# Autodesk Inventor assembly: Assembly1
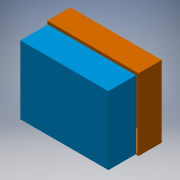
[picture p0: Inventor's stored thumbnail of the model, 180x180]
Saved by Autodesk Inventor 2016 (Build 200138000, 138)
## iProperties
Created: 2016-02-20
Part Number: Assembly1
Document SubType Name: Assembly
Designer: Róbert
Author: Róbert
## Documents named in this file (5)
- C:\Users\Róbert\Desktop\Mechatronics-2016.git\trunk\Inventor\Assembly1.iam
- C:\Users\Róbert\Desktop\Mechatronics-2016.git\trunk\Inventor\veggur_lok.ipt
- C:\Users\Róbert\Desktop\Mechatronics-2016.git\trunk\Inventor\toppur.ipt
- C:\Users\Róbert\Desktop\Mechatronics-2016.git\trunk\Inventor\botn.ipt
- C:\Users\Róbert\Desktop\Mechatronics-2016.git\trunk\Inventor\veggur.ipt
## Components (4 placed, 4 different names)
1. veggur_lok:1 — Mate:1, Flush:1, Flush:2, Mate:3
2. toppur:1 — Mate:1, Flush:1, Flush:2
3. botn:1 — Mate:2, Flush:3, Flush:4
4. veggur:1 — Mate:2, Flush:3, Flush:4, Mate:3
## Relationships (7: Flush 4, Mate 3)
- Mate:1: veggur_lok:1 ↔ toppur:1
- Flush:1: veggur_lok:1 ↔ toppur:1
- Flush:2: veggur_lok:1 ↔ toppur:1
- Mate:2: botn:1 ↔ veggur:1
- Flush:3: botn:1 ↔ veggur:1
- Flush:4: botn:1 ↔ veggur:1
- Mate:3: veggur_lok:1 ↔ veggur:1
